# Autodesk Inventor assembly: om_Interior_2.0
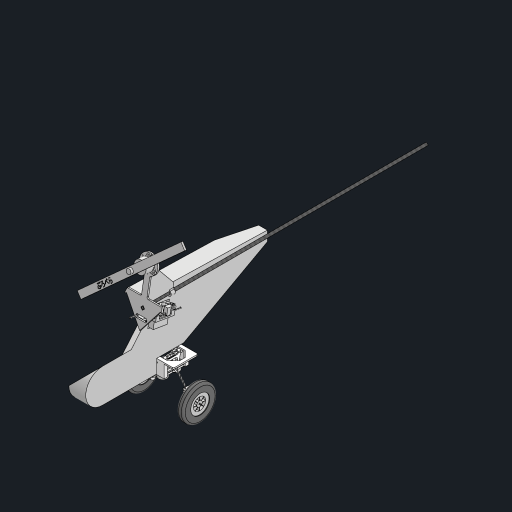
[picture p0: Inventor's stored thumbnail of the model, 512x512]
Saved by Autodesk Inventor 2023 (Build 270158000, 158)
## iProperties
Created: 2022-06-22
Part Number: om_Interior_2.0
Document SubType Name: Assembly
Designer: legot
Author: legot
## Documents named in this file (8)
- C:\Users\legot\OneDrive\ドキュメント\Inventor\HIKOSAPO\OM\om_Interior_2.0.iam
- C:\Users\legot\OneDrive\ドキュメント\Inventor\HIKOSAPO\OM\om_Body_2.0.ipt
- C:\Users\legot\OneDrive\ドキュメント\Inventor\HIKOSAPO\OM\om_MotorMount_2.0.ipt
- C:\Users\legot\OneDrive\ドキュメント\Inventor\HIKOSAPO\Drop\om_Drop.iam
- C:\Users\legot\OneDrive\ドキュメント\Inventor\HIKOSAPO\public_parts\MainRod.ipt
- C:\Users\legot\OneDrive\ドキュメント\Inventor\HIKOSAPO\public_parts\MainMotor.ipt
- C:\Users\legot\OneDrive\ドキュメント\Inventor\HIKOSAPO\public_parts\Propeller.ipt
- C:\Users\legot\OneDrive\ドキュメント\Inventor\HIKOSAPO\Gear\GearV1.iam
## Components (7 placed, 7 different names)
1. om_Body_2.0:1 — メイト:1, メイト:2, メイト:3, メイト:4, メイト:5, メイト:6, メイト:7, メイト:8, フラッシュ:2, メイト:10, メイト:11
2. om_MotorMount_2.0:1 — メイト:1, フラッシュ:1, メイト:7, メイト:8, 挿入:1, メイト:9
3. om_Drop:1 [sub-assembly] — メイト:2, メイト:3, メイト:4
4. MainRod:1 — フラッシュ:1, メイト:5, メイト:6
5. MainMotor:1 — 挿入:1, メイト:9, 挿入:2
6. Propeller:1 — 挿入:2
7. GearV1:1 [sub-assembly] — フラッシュ:2, メイト:10, メイト:11
## Relationships (15: Mate 11, Flush 2, Insert 2)
- メイト:1 [Mate]: om_Body_2.0:1 ↔ om_MotorMount_2.0:1
- メイト:2 [Mate]: om_Body_2.0:1 ↔ om_Drop:1
- メイト:3 [Mate]: om_Body_2.0:1 ↔ om_Drop:1
- メイト:4 [Mate]: om_Body_2.0:1 ↔ om_Drop:1
- フラッシュ:1 [Flush]: om_MotorMount_2.0:1 ↔ MainRod:1
- メイト:5 [Mate]: om_Body_2.0:1 ↔ MainRod:1
- メイト:6 [Mate]: om_Body_2.0:1 ↔ MainRod:1
- メイト:7 [Mate]: om_Body_2.0:1 ↔ om_MotorMount_2.0:1
- メイト:8 [Mate]: om_Body_2.0:1 ↔ om_MotorMount_2.0:1
- 挿入:1 [Insert]: om_MotorMount_2.0:1 ↔ MainMotor:1
- メイト:9 [Mate]: om_MotorMount_2.0:1 ↔ MainMotor:1
- 挿入:2 [Insert]: MainMotor:1 ↔ Propeller:1
- フラッシュ:2 [Flush]: om_Body_2.0:1 ↔ GearV1:1
- メイト:10 [Mate]: om_Body_2.0:1 ↔ GearV1:1
- メイト:11 [Mate]: om_Body_2.0:1 ↔ GearV1:1
